# Autodesk Inventor assembly: rico
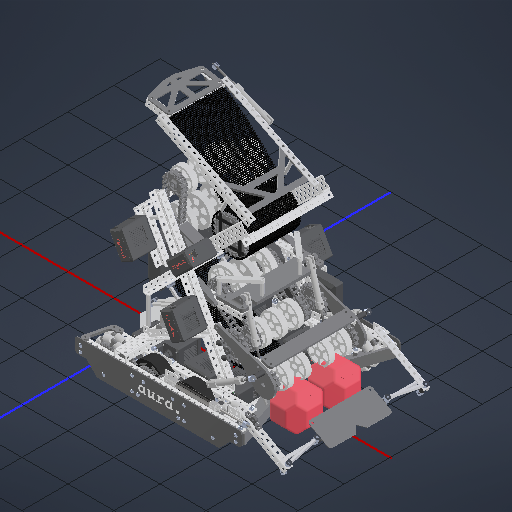
[picture p0: Inventor's stored thumbnail of the model, 512x512]
Saved by Autodesk Inventor 2025.2 (Build 292293000, 293)
## iProperties
Created: 2025-12-05
Part Number: rico
Document SubType Name: Assembly
Designer: cloudy
Author: cloudy
## Documents named in this file (14)
- C:\Users\cloudy\Documents\GitHub\aura-cad\15\rico.iam
- C:\Users\cloudy\Documents\GitHub\aura-cad\15\Drivetrain\!drivetrain.iam
- C:\Users\cloudy\Documents\GitHub\aura-cad\15\structure.iam
- C:\Users\cloudy\Documents\GitHub\aura-cad\15\intake.iam
- C:\Users\cloudy\Documents\GitHub\aura-cad\15\hood.iam
- C:\Users\cloudy\Documents\GitHub\aura-cad\15\25 stroke 10 bore\CJ2D10-25Z(0_0).iam
- C:\Users\cloudy\Documents\GitHub\aura-cad\!lib\Motion\Shaft LS\Shaft Collar Metal\Shaft Collar No Screw.iam
- C:\Users\cloudy\Documents\GitHub\aura-cad\!lib\Motion\Shaft LS\Shaft Collar Metal.iam
- C:\Users\cloudy\Documents\GitHub\aura-cad\15\meshramp.ipt
- C:\Users\cloudy\Documents\GitHub\aura-cad\15\scraper.iam
- C:\Users\cloudy\Documents\GitHub\aura-cad\!lib\Structure\Standoff\Standoff 6.00.ipt
- C:\Users\cloudy\Documents\GitHub\aura-cad\!lib\Structure\Standoff.ipt
- C:\Users\cloudy\Downloads\cube\cube\cube.ipt
- C:\Users\cloudy\Documents\GitHub\aura-cad\!lib\Miscellaneous\iw_metal_02.bmp
## Components (17 placed, 10 different names)
1. !drivetrain:1 [sub-assembly] — Insert:1, Mate:1, Insert:10, Mate:8, Insert:17
2. structure:1 [sub-assembly] — Insert:1, Mate:1, Insert:2, Insert:5, Flush:2, Mate:9, Mate:10, Insert:18
3. intake:1 [sub-assembly] — Insert:2, Insert:11, Insert:14
4. hood:1 [sub-assembly] — Insert:5
5. meshramp:1 — Flush:2
6. scraper:1 [sub-assembly] — Insert:10, Mate:8
7. CJ2D10-25Z(0_0):1 [sub-assembly] — Insert:12, Mate:9
8. Shaft Collar No Screw:2 [sub-assembly] — Insert:11, Insert:12
9. CJ2D10-25Z(0_0):2 [sub-assembly] — Mate:10
10. Shaft Collar No Screw:3 [sub-assembly] — Insert:14
11. Shaft Collar No Screw:4 [sub-assembly] — Insert:15, Insert:18
12. Shaft Collar No Screw:5 [sub-assembly] — Insert:15, Mate:11
13. Shaft Collar No Screw:6 [sub-assembly] — Insert:17
14. Shaft Collar No Screw:7 [sub-assembly] — Insert:19
15. Standoff 6.00:1 — Insert:19, Mate:11
16. cube:1
17. cube:2
## Relationships (19: Insert 13, Mate 5, Flush 1)
- Insert:1: !drivetrain:1 ↔ structure:1
- Mate:1: !drivetrain:1 ↔ structure:1
- Insert:2: structure:1 ↔ intake:1
- Insert:5 (12.7 mm): structure:1 ↔ hood:1
- Flush:2: structure:1 ↔ meshramp:1
- Insert:10 (12.7 mm): !drivetrain:1 ↔ scraper:1
- Mate:8: !drivetrain:1 ↔ scraper:1
- Insert:11 (20.6375 mm): intake:1 ↔ Shaft Collar No Screw:2
- Insert:12: CJ2D10-25Z(0_0):1 ↔ Shaft Collar No Screw:2
- Mate:9: structure:1 ↔ CJ2D10-25Z(0_0):1
- [Insert]: CJ2D10-25Z(0_0):2 ↔ Shaft Collar No Screw:3
- Insert:14 (20.6375 mm): intake:1 ↔ Shaft Collar No Screw:3
- Mate:10: structure:1 ↔ CJ2D10-25Z(0_0):2
- Insert:15: Shaft Collar No Screw:4 ↔ Shaft Collar No Screw:5
- [Insert]: Shaft Collar No Screw:6 ↔ Shaft Collar No Screw:7
- Insert:17 (12.7 mm): !drivetrain:1 ↔ Shaft Collar No Screw:6
- Insert:18 (15.875 mm): structure:1 ↔ Shaft Collar No Screw:4
- Insert:19: Shaft Collar No Screw:7 ↔ Standoff 6.00:1
- Mate:11: Shaft Collar No Screw:5 ↔ Standoff 6.00:1
## Named parameters: d25_d23 = 0 mm, d29_d28 = 0 mm
